# Autodesk Inventor assembly: Grabber Tool
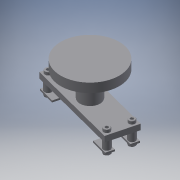
[picture p0: Inventor's stored thumbnail of the model, 180x180]
Saved by Autodesk Inventor 2019.4 (Build 234330000, 330)
## iProperties
Created: 2020-12-03
Part Number: Grabber Tool
Document SubType Name: Assembly
Designer: caleb
Author: caleb
## Documents named in this file (8)
- C:\Users\cfang\Desktop\nebraska-silicon-lab\CAD\ETL\Module Assembly\Grabber Tool\Grabber Tool.iam
- C:\Users\cfang\Desktop\nebraska-silicon-lab\CAD\ETL\Module Assembly\Grabber Tool\Grabber Base.ipt
- C:\Users\cfang\Desktop\nebraska-silicon-lab\CAD\ETL\Module Assembly\Grabber Tool\Grabber Platform.ipt
- C:\Users\cfang\Desktop\nebraska-silicon-lab\CAD\ETL\Module Assembly\Grabber Tool\Standoff.ipt
- C:\Users\cfang\Desktop\nebraska-silicon-lab\CAD\ETL\Module Assembly\Grabber Tool\Picker Strip.ipt
- C:\Users\cfang\Desktop\nebraska-silicon-lab\CAD\ETL\Module Assembly\Grabber Tool\92290A761_TYPE 316 SS SOCKET HEAD CAP SCREW.ipt
- C:\Users\cfang\Desktop\nebraska-silicon-lab\CAD\ETL\Module Assembly\Grabber Tool\92125A130_TYPE 18-8 SS FLAT-HEAD SOCKET CAP SCREW.ipt
- C:\Users\cfang\Desktop\nebraska-silicon-lab\CAD\ETL\Module Assembly\Grabber Tool\91828A211_TYPE 18-8 STAINLESS STEEL HEX NUT.ipt
## Components (22 placed, 7 different names)
1. Grabber Base:1 — Insert:1, Mate:1
2. Grabber Platform:1 — Insert:1, Mate:1, Insert:2, Insert:3, Insert:4, Insert:5, Angle:1, Angle:2, Angle:3, Angle:4, Insert:10, Insert:11, Insert:12, Insert:13, Insert:14, Insert:15, Insert:16, Insert:17
3. Standoff:1 — Insert:3, Insert:8
4. Standoff:2 — Insert:2, Insert:9
5. Standoff:3 — Insert:5, Insert:7
6. Standoff:4 — Insert:4, Insert:6
7. Picker Strip:1 — Insert:6, Angle:1, Insert:18
8. Picker Strip:2 — Insert:7, Angle:2, Insert:19
9. Picker Strip:3 — Insert:9, Angle:4, Insert:20
10. Picker Strip:4 — Insert:8, Angle:3, Insert:21
11. 92290A761_TYPE 316 SS SOCKET HEAD CAP SCREW:1 — Insert:11
12. 92290A761_TYPE 316 SS SOCKET HEAD CAP SCREW:2 — Insert:10
13. 92290A761_TYPE 316 SS SOCKET HEAD CAP SCREW:3 — Insert:13
14. 92290A761_TYPE 316 SS SOCKET HEAD CAP SCREW:4 — Insert:12
15. 92125A130_TYPE 18-8 SS FLAT-HEAD SOCKET CAP SCREW:1 — Insert:15
16. 92125A130_TYPE 18-8 SS FLAT-HEAD SOCKET CAP SCREW:2 — Insert:14
17. 92125A130_TYPE 18-8 SS FLAT-HEAD SOCKET CAP SCREW:3 — Insert:17
18. 92125A130_TYPE 18-8 SS FLAT-HEAD SOCKET CAP SCREW:4 — Insert:16
19. 91828A211_TYPE 18-8 STAINLESS STEEL HEX NUT:1 — Insert:19
20. 91828A211_TYPE 18-8 STAINLESS STEEL HEX NUT:2 — Insert:18
21. 91828A211_TYPE 18-8 STAINLESS STEEL HEX NUT:3 — Insert:21
22. 91828A211_TYPE 18-8 STAINLESS STEEL HEX NUT:4 — Insert:20
## Relationships (26: Insert 21, Angle 4, Mate 1)
- Insert:1: Grabber Base:1 ↔ Grabber Platform:1
- Mate:1: Grabber Base:1 ↔ Grabber Platform:1
- Insert:2: Grabber Platform:1 ↔ Standoff:2
- Insert:3: Grabber Platform:1 ↔ Standoff:1
- Insert:4: Grabber Platform:1 ↔ Standoff:4
- Insert:5: Grabber Platform:1 ↔ Standoff:3
- Insert:6: Standoff:4 ↔ Picker Strip:1
- Insert:7: Standoff:3 ↔ Picker Strip:2
- Angle:1 (0 deg): Grabber Platform:1 ↔ Picker Strip:1
- Angle:2 (0 deg): Grabber Platform:1 ↔ Picker Strip:2
- Insert:8: Standoff:1 ↔ Picker Strip:4
- Insert:9: Standoff:2 ↔ Picker Strip:3
- Angle:3 (0 deg): Grabber Platform:1 ↔ Picker Strip:4
- Angle:4 (0 deg): Grabber Platform:1 ↔ Picker Strip:3
- Insert:10: Grabber Platform:1 ↔ 92290A761_TYPE 316 SS SOCKET HEAD CAP SCREW:2
- Insert:11: Grabber Platform:1 ↔ 92290A761_TYPE 316 SS SOCKET HEAD CAP SCREW:1
- Insert:12: Grabber Platform:1 ↔ 92290A761_TYPE 316 SS SOCKET HEAD CAP SCREW:4
- Insert:13: Grabber Platform:1 ↔ 92290A761_TYPE 316 SS SOCKET HEAD CAP SCREW:3
- Insert:14: Grabber Platform:1 ↔ 92125A130_TYPE 18-8 SS FLAT-HEAD SOCKET CAP SCREW:2
- Insert:15: Grabber Platform:1 ↔ 92125A130_TYPE 18-8 SS FLAT-HEAD SOCKET CAP SCREW:1
- Insert:16: Grabber Platform:1 ↔ 92125A130_TYPE 18-8 SS FLAT-HEAD SOCKET CAP SCREW:4
- Insert:17: Grabber Platform:1 ↔ 92125A130_TYPE 18-8 SS FLAT-HEAD SOCKET CAP SCREW:3
- Insert:18: Picker Strip:1 ↔ 91828A211_TYPE 18-8 STAINLESS STEEL HEX NUT:2
- Insert:19: Picker Strip:2 ↔ 91828A211_TYPE 18-8 STAINLESS STEEL HEX NUT:1
- Insert:20: Picker Strip:3 ↔ 91828A211_TYPE 18-8 STAINLESS STEEL HEX NUT:4
- Insert:21: Picker Strip:4 ↔ 91828A211_TYPE 18-8 STAINLESS STEEL HEX NUT:3
